# Autodesk Inventor assembly: Assembly
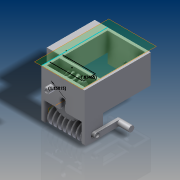
[picture p0: Inventor's stored thumbnail of the model, 180x180]
Saved by Autodesk Inventor 2015 SP1 (Build 190203100, 203)
## iProperties
Created: 2015-04-25
Part Number: Assembly
Document SubType Name: Assembly
Designer: Trevor
Author: Trevor
## Documents named in this file (6)
- C:\Users\Trevor\Google Drive\Classwork\6.S079\Project\6.s079-musicbox\CAD\Assembly.iam
- C:\Users\Trevor\Google Drive\Classwork\6.S079\Project\6.s079-musicbox\CAD\Assembly\Design Accelerator\Worm Gears1.iam
- C:\Users\Trevor\Google Drive\Classwork\6.S079\Project\6.s079-musicbox\CAD\Assembly\Design Accelerator\Worm1.ipt
- C:\Users\Trevor\Google Drive\Classwork\6.S079\Project\6.s079-musicbox\CAD\Crank.ipt
- C:\Users\Trevor\Google Drive\Classwork\6.S079\Project\6.s079-musicbox\CAD\Box.ipt
- C:\Users\Trevor\Google Drive\Classwork\6.S079\Project\6.s079-musicbox\CAD\axle.ipt
## Components (4 placed, 4 different names)
1. Worm Gears:1 [sub-assembly] — Mate:4, Insert:1, Rotation:1
2. Crank:1 — Rotation:1
3. Box:1 — Mate:4, Insert:1
4. axle:1
## Relationships (3: Mate 1, Insert 1, RelateRotation 1)
- Mate:4: Worm Gears:1 ↔ Box:1
- Insert:1: Worm Gears:1 ↔ Box:1
- Rotation:1 [RelateRotation] (1 ul): Worm Gears:1 ↔ Crank:1
## Named parameters: l_key = 6.73519 mm, d_key = 6.35 mm
